# Autodesk Inventor assembly: 二連趕
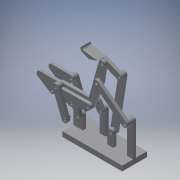
[picture p0: Inventor's stored thumbnail of the model, 180x180]
Saved by Autodesk Inventor 2017 (Build 210142000, 142)
## iProperties
Part Number: 二連趕
Material: 一般
Document SubType Name: Assembly
Designer: 士正
Author: 士正
## Documents named in this file (12)
- C:\Users\士正\Desktop\git\二連趕.iam
- C:\Users\士正\Desktop\git\實體2.ipt
- C:\Users\士正\Desktop\git\實體1.ipt
- C:\Users\士正\Desktop\git\實體3.ipt
- C:\Users\士正\Desktop\git\實體4.ipt
- C:\Users\士正\Desktop\git\實體5.ipt
- C:\Users\士正\Desktop\git\實體6.ipt
- C:\Users\士正\Desktop\git\實體7.ipt
- C:\Users\士正\Desktop\git\實體8.ipt
- C:\Users\士正\Desktop\git\實體9.ipt
- C:\Users\士正\Desktop\git\實體11.ipt
- C:\Users\士正\Desktop\git\pin.ipt
## Components (27 placed, 11 different names)
1. 實體2:1 — 貼合:6, 貼合:15, 貼合:26, 貼合:41, 齊平:11, 貼合:43, 齊平:13
2. 實體1:1 — 貼合:3, 貼合:8, 貼合:12, 貼合:18, 貼合:21, 貼合:24, 貼合:39, 齊平:9
3. 實體3:1 — 貼合:5, 貼合:13, 貼合:19, 貼合:32, 貼合:40, 齊平:10
4. 實體4:1 — 貼合:9, 貼合:11, 貼合:30, 貼合:31
5. 實體5:1 — 貼合:10, 貼合:11, 貼合:31, 貼合:35, 齊平:5
6. 實體6:1 — 貼合:4, 貼合:7, 貼合:33, 齊平:3, 貼合:47
7. 實體7:1 — 貼合:17, 貼合:20, 貼合:27, 貼合:28, 貼合:45, 齊平:15, 貼合:46, 齊平:16
8. 實體8:1 — 貼合:18, 貼合:19, 貼合:20, 貼合:23, 貼合:24, 貼合:27
9. 實體9:1 — 貼合:7, 貼合:8, 貼合:10, 貼合:22, 貼合:23, 貼合:36, 齊平:6, 貼合:37, 齊平:7, 貼合:47
10. 實體11:1 — 貼合:1, 齊平:1, 齊平:2, 貼合:3, 貼合:4, 貼合:5, 貼合:6, 貼合:9, 貼合:16, 貼合:21, 貼合:30, 貼合:32, 貼合:34, 齊平:4
11. 實體2:2 — 貼合:16, 貼合:17, 貼合:28
12. 實體8:2 — 貼合:12, 貼合:13, 貼合:14, 貼合:22, 貼合:25, 貼合:38, 齊平:8, 貼合:42, 齊平:12
13. 實體7:2 — 貼合:14, 貼合:15, 貼合:25, 貼合:26, 貼合:44, 齊平:14
14. pin:1 — 貼合:37, 齊平:7
15. pin:2 — 貼合:38, 齊平:8
16. pin:3 — 貼合:36, 齊平:6
17. pin:5 — 貼合:45, 齊平:15
18. pin:6 — 貼合:42, 齊平:12
19. pin:7 — 貼合:41, 齊平:11
20. pin:8 — 貼合:35, 齊平:5
21. pin:9 — 貼合:34, 齊平:4
22. pin:10 — 貼合:33, 齊平:3
23. pin:11 — 貼合:39, 齊平:9
24. pin:12 — 貼合:40, 齊平:10
25. pin:13 — 貼合:43, 齊平:13
26. pin:14 — 貼合:44, 齊平:14
27. pin:15 — 貼合:46, 齊平:16
## Relationships (61: Mate 45, Flush 16)
- 貼合:1 [Mate]: 實體11:1
- 齊平:1 [Flush]: 實體11:1
- 齊平:2 [Flush]: 實體11:1
- 貼合:3 [Mate]: 實體1:1 ↔ 實體11:1
- 貼合:4 [Mate]: 實體6:1 ↔ 實體11:1
- 貼合:5 [Mate]: 實體3:1 ↔ 實體11:1
- 貼合:6 [Mate]: 實體2:1 ↔ 實體11:1
- 貼合:7 [Mate]: 實體6:1 ↔ 實體9:1
- 貼合:8 [Mate]: 實體1:1 ↔ 實體9:1
- 貼合:9 [Mate]: 實體4:1 ↔ 實體11:1
- 貼合:10 [Mate]: 實體5:1 ↔ 實體9:1
- 貼合:11 [Mate]: 實體4:1 ↔ 實體5:1
- 貼合:12 [Mate]: 實體1:1 ↔ 實體8:2
- 貼合:13 [Mate]: 實體3:1 ↔ 實體8:2
- 貼合:14 [Mate]: 實體8:2 ↔ 實體7:2
- 貼合:15 [Mate]: 實體2:1 ↔ 實體7:2
- 貼合:16 [Mate]: 實體11:1 ↔ 實體2:2
- 貼合:17 [Mate]: 實體7:1 ↔ 實體2:2
- 貼合:18 [Mate]: 實體1:1 ↔ 實體8:1
- 貼合:19 [Mate]: 實體3:1 ↔ 實體8:1
- 貼合:20 [Mate]: 實體7:1 ↔ 實體8:1
- 貼合:21 [Mate]: 實體1:1 ↔ 實體11:1
- 貼合:22 [Mate]: 實體9:1 ↔ 實體8:2
- 貼合:23 [Mate]: 實體8:1 ↔ 實體9:1
- 貼合:24 [Mate]: 實體1:1 ↔ 實體8:1
- 貼合:25 [Mate]: 實體8:2 ↔ 實體7:2
- 貼合:26 [Mate]: 實體2:1 ↔ 實體7:2
- 貼合:27 [Mate]: 實體7:1 ↔ 實體8:1
- 貼合:28 [Mate]: 實體7:1 ↔ 實體2:2
- 貼合:30 [Mate]: 實體4:1 ↔ 實體11:1
- 貼合:31 [Mate]: 實體4:1 ↔ 實體5:1
- 貼合:32 [Mate]: 實體3:1 ↔ 實體11:1
- 貼合:33 [Mate]: 實體6:1 ↔ pin:10
- 齊平:3 [Flush]: 實體6:1 ↔ pin:10
- 貼合:34 [Mate]: 實體11:1 ↔ pin:9
- 齊平:4 [Flush]: 實體11:1 ↔ pin:9
- 貼合:35 [Mate]: 實體5:1 ↔ pin:8
- 齊平:5 [Flush]: 實體5:1 ↔ pin:8
- 貼合:36 [Mate]: 實體9:1 ↔ pin:3
- 齊平:6 [Flush]: 實體9:1 ↔ pin:3
- 貼合:37 [Mate]: 實體9:1 ↔ pin:1
- 齊平:7 [Flush]: 實體9:1 ↔ pin:1
- 貼合:38 [Mate]: 實體8:2 ↔ pin:2
- 齊平:8 [Flush]: 實體8:2 ↔ pin:2
- 貼合:39 [Mate]: 實體1:1 ↔ pin:11
- 齊平:9 [Flush]: 實體1:1 ↔ pin:11
- 貼合:40 [Mate]: 實體3:1 ↔ pin:12
- 齊平:10 [Flush]: 實體3:1 ↔ pin:12
- 貼合:41 [Mate]: 實體2:1 ↔ pin:7
- 齊平:11 [Flush]: 實體2:1 ↔ pin:7
- 貼合:42 [Mate]: 實體8:2 ↔ pin:6
- 齊平:12 [Flush]: 實體8:2 ↔ pin:6
- 貼合:43 [Mate]: 實體2:1 ↔ pin:13
- 齊平:13 [Flush]: 實體2:1 ↔ pin:13
- 貼合:44 [Mate]: 實體7:2 ↔ pin:14
- 齊平:14 [Flush]: 實體7:2 ↔ pin:14
- 貼合:45 [Mate]: 實體7:1 ↔ pin:5
- 齊平:15 [Flush]: 實體7:1 ↔ pin:5
- 貼合:46 [Mate]: 實體7:1 ↔ pin:15
- 齊平:16 [Flush]: 實體7:1 ↔ pin:15
- 貼合:47 [Mate]: 實體6:1 ↔ 實體9:1
